# Autodesk Inventor assembly: AlarmClock
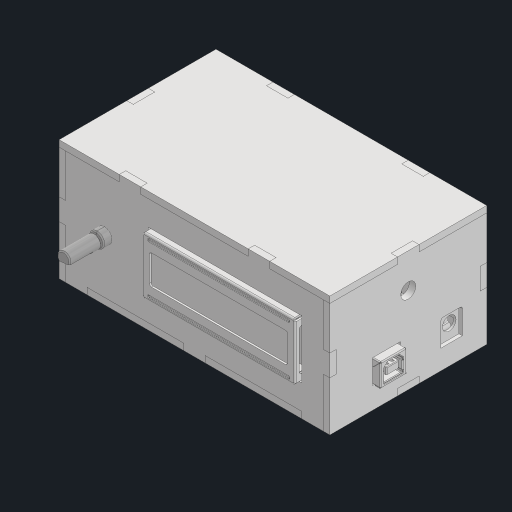
[picture p0: Inventor's stored thumbnail of the model, 512x512]
Saved by Autodesk Inventor 2023 (Build 270158000, 158)
## iProperties
Created: 2024-07-21
Part Number: AlarmClock
Document SubType Name: Assembly
Designer: Orsted
Author: Orsted
## Documents named in this file (10)
- E:\personal\project\Design\AlarmClock.iam
- C:\Users\Orsted\Downloads\Rotary Encoder -  ODG\sw2017 model\KY-040 Rotary Encoder.iam
- C:\Users\Orsted\Downloads\16-x-2-lcd-display-module.snapshot.1\LCD.iam
- C:\Users\Orsted\Downloads\arduino-uno-r3-1.snapshot.5\arduino uno.iam
- E:\personal\project\Design\Front-panel.ipt
- E:\personal\project\Design\Bottom.ipt
- E:\personal\project\Design\left.ipt
- E:\personal\project\Design\right.ipt
- E:\personal\project\Design\back.ipt
- E:\personal\project\Design\top.ipt
## Components (9 placed, 9 different names)
1. KY-040 Rotary Encoder:2 [sub-assembly] — Mate:3, Angle:1, Mate:4
2. LCD:1 [sub-assembly] — Mate:1, Mate:2, Flush:1
3. arduino uno:1 [sub-assembly] — Mate:8, Mate:9
4. Front-panel:1 — Mate:1, Mate:2, Flush:1, Mate:3, Angle:1, Mate:4, Mate:5, Flush:2, Flush:3, Mate:9, Flush:11, Flush:13, Flush:14
5. Bottom:1 — Mate:5, Flush:2, Flush:3, Mate:8, Mate:14, Flush:7, Flush:10, Flush:12
6. left:1 — Flush:12, Flush:13, Mate:15, Flush:15
7. right:1 — Flush:10, Flush:11
8. back:1 — Mate:14, Flush:7
9. top:1 — Mate:15, Flush:14, Flush:15
## Relationships (20: Flush 10, Mate 9, Angle 1)
- Mate:1 (0.1 mm): LCD:1 ↔ Front-panel:1
- Mate:2 (0.1 mm): LCD:1 ↔ Front-panel:1
- Flush:1 (-3 mm): LCD:1 ↔ Front-panel:1
- Mate:3: KY-040 Rotary Encoder:2 ↔ Front-panel:1
- Angle:1 (0 deg): KY-040 Rotary Encoder:2 ↔ Front-panel:1
- Mate:4: KY-040 Rotary Encoder:2 ↔ Front-panel:1
- Mate:5: Front-panel:1 ↔ Bottom:1
- Flush:2: Front-panel:1 ↔ Bottom:1
- Flush:3: Front-panel:1 ↔ Bottom:1
- Mate:8 (5 mm): arduino uno:1 ↔ Bottom:1
- Mate:9 (8 mm): arduino uno:1 ↔ Front-panel:1
- Mate:14: Bottom:1 ↔ back:1
- Flush:7: Bottom:1 ↔ back:1
- Flush:10: Bottom:1 ↔ right:1
- Flush:11: Front-panel:1 ↔ right:1
- Flush:12: Bottom:1 ↔ left:1
- Flush:13: Front-panel:1 ↔ left:1
- Mate:15: left:1 ↔ top:1
- Flush:14: Front-panel:1 ↔ top:1
- Flush:15: left:1 ↔ top:1
